# Autodesk Inventor assembly: dummy_expansion_ring_assembly
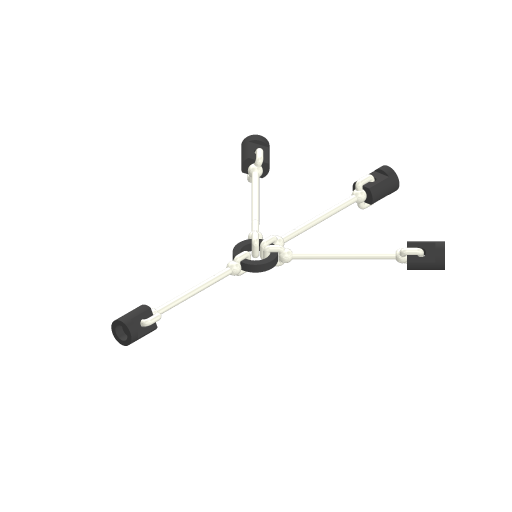
[picture p0: Inventor's stored thumbnail of the model, 512x512]
Saved by Autodesk Inventor 2024.3 (Build 283343000, 343)
## iProperties
Created: 2024-09-12
Part Number: dummy_expansion_ring_assembly
Document SubType Name: Assembly
Designer: gihyeok2
Author: gihyeok2
## Documents named in this file (3)
- C:\Users\gihyeok2\Desktop\New folder\component\mckibben_pam_module\dummy_expansion_ring_assembly.iam
- C:\Users\gihyeok2\Desktop\New folder\component\mckibben_pam_module\dummy_anchor_end_3.0mm_with_string.ipt
- C:\Users\gihyeok2\Desktop\New folder\component\mckibben_pam_module\dummy_expansion_ring_4.8mm_with_string.ipt
## Components (5 placed, 2 different names)
1. dummy_expansion_ring_4.8mm_with_string:1 — Mate:1, Mate:2, Mate:3, Mate:4, Mate:5, Mate:6, Mate:7, Mate:8
2. dummy_anchor_end_3.0mm_with_string:1 — Mate:1, Mate:5
3. dummy_anchor_end_3.0mm_with_string:2 — Mate:3, Mate:6
4. dummy_anchor_end_3.0mm_with_string:3 — Mate:2, Mate:8
5. dummy_anchor_end_3.0mm_with_string:4 — Mate:4, Mate:7
## Relationships (8: Mate 8)
- Mate:1: dummy_expansion_ring_4.8mm_with_string:1 ↔ dummy_anchor_end_3.0mm_with_string:1
- Mate:2: dummy_expansion_ring_4.8mm_with_string:1 ↔ dummy_anchor_end_3.0mm_with_string:3
- Mate:3: dummy_expansion_ring_4.8mm_with_string:1 ↔ dummy_anchor_end_3.0mm_with_string:2
- Mate:4: dummy_expansion_ring_4.8mm_with_string:1 ↔ dummy_anchor_end_3.0mm_with_string:4
- Mate:5: dummy_expansion_ring_4.8mm_with_string:1 ↔ dummy_anchor_end_3.0mm_with_string:1
- Mate:6: dummy_expansion_ring_4.8mm_with_string:1 ↔ dummy_anchor_end_3.0mm_with_string:2
- Mate:7: dummy_expansion_ring_4.8mm_with_string:1 ↔ dummy_anchor_end_3.0mm_with_string:4
- Mate:8: dummy_expansion_ring_4.8mm_with_string:1 ↔ dummy_anchor_end_3.0mm_with_string:3
